# Autodesk Inventor assembly: tower1
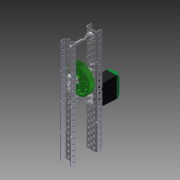
[picture p0: Inventor's stored thumbnail of the model, 180x180]
Saved by Autodesk Inventor 2014 SP1 (Build 180222100, 222)
## iProperties
Created: 2013-08-29
Part Number: tower1
Document SubType Name: Assembly
Designer: Ryan
Author: Ryan
## Documents named in this file (19)
- C:\Users\Ryan\Desktop\sw\toss up 1st A bot\toss up tower\tower1.iam
- C:\Users\Ryan\Desktop\sw\lib\Aperture VEX CAD Library\Metal\C Channel\2 x 20.ipt
- C:\Users\Ryan\Desktop\sw\lib\Aperture VEX CAD Library\Bearing Blocks\Bearing Block with screws.iam
- C:\Users\Ryan\Desktop\sw\lib\Aperture VEX CAD Library\Hardware\8-32\8-32_.375.ipt
- C:\Users\Ryan\Desktop\sw\lib\Aperture VEX CAD Library\Shaft\2 inch Shaft.ipt
- C:\Users\Ryan\Desktop\sw\lib\Aperture VEX CAD Library\Gears\High Strength Gears\60 Tooth Round Insert.iam
- C:\Users\Ryan\Desktop\sw\lib\Aperture VEX CAD Library\Gears\High Strength Gears\HS-GEAR-12TOOTH.ipt
- C:\Users\Ryan\Desktop\sw\lib\Super Sonic Sparks VEX CAD Library\Motors & Sensors\2-Wire Motor 393-Without Wire.iam
- C:\Users\Ryan\Desktop\sw\lib\Aperture VEX CAD Library\Bearing Blocks\Bearing Block.ipt
- C:\Users\Ryan\Desktop\sw\lib\Aperture VEX CAD Library\Hardware\6-32\6-32_.500.ipt
- C:\Users\Ryan\Desktop\sw\lib\Aperture VEX CAD Library\Shaft\3 inch Shaft.ipt
- C:\Users\Ryan\Desktop\sw\lib\Aperture VEX CAD Library\Spacers\SPACER-0500-0125.ipt
- C:\Users\Ryan\Desktop\sw\lib\Aperture VEX CAD Library\Spacers\SPACER-0500-0500.ipt
- C:\Users\Ryan\Desktop\sw\lib\Aperture VEX CAD Library\Spacers\SPACER-0500-0250.ipt
- C:\Users\Ryan\Desktop\sw\lib\Aperture VEX CAD Library\Hardware\Shaft Collar.ipt
- C:\Users\Ryan\Desktop\sw\lib\Aperture VEX CAD Library\Metal\0.5x12.5 inch Beam.ipt
- C:\Users\Ryan\Desktop\sw\lib\Imported Components\8-32 nylock\8-32 nylock.ipt
- C:\Users\Ryan\Desktop\sw\lib\Aperture VEX CAD Library\Hardware\8-32\8-32_1.500.ipt
- C:\Users\Ryan\Desktop\sw\lib\Aperture VEX CAD Library\Standoffs\BEAM-1000.ipt
## Components (31 placed, 18 different names)
1. 2 x 20:1 — Flush:1, Flush:3, Mate:33, Flush:4, Mate:87, Mate:88, Mate:89, Mate:90, Mate:91, Mate:98, Mate:101, Mate:102, Mate:103, Mate:104, Mate:117, Flush:7, Flush:8, Flush:10, Mate:131, Mate:134
2. 2 x 20:2 — Flush:4, Mate:34, Mate:35, Mate:40, Mate:41, Mate:44, Flush:9, Flush:10, Mate:120, Mate:127, Mate:128, Mate:129, Mate:141
3. 2-Wire Motor 393-Without Wire:1 [sub-assembly] — Mate:34, Mate:45, Mate:46, Mate:50
4. 0.5x12.5 inch Beam:1 — Mate:117, Flush:7, Flush:8, Flush:9
5. Bearing Block with screws:2 [sub-assembly] — Mate:100, Mate:101, Mate:102, Mate:103, Mate:104, Mate:105
6. 3 inch Shaft:1 — Mate:50, Mate:51, Mate:52, Mate:53, Mate:54
7. HS-GEAR-12TOOTH:1 — Rotation:1, Mate:53, Mate:54, Mate:106, Mate:118
8. Bearing Block:1 — Mate:35, Mate:36, Mate:37, Mate:42, Mate:43, Mate:51, Mate:52, Mate:107, Mate:108
9. 6-32_.500:1 — Mate:36, Mate:37, Mate:40, Mate:41, Mate:46
10. 6-32_.500:2 — Mate:42, Mate:43, Mate:44, Mate:45
11. SPACER-0500-0250:1 — Mate:100, Mate:105, Mate:106
12. SPACER-0500-0250:2 — Mate:107, Mate:108, Mate:114, Mate:115
13. SPACER-0500-0125:3 — Mate:114, Mate:115, Mate:116
14. Shaft Collar:1 — Mate:116, Mate:118
15. 8-32 nylock:1 — Mate:126, Mate:127, Mate:128, Mate:130
16. 8-32_1.500:1 — Mate:129, Mate:130, Mate:132, Mate:137, Mate:140
17. 8-32_.375:19 — Mate:131, Mate:132, Mate:133
18. BEAM-1000:1 — Mate:133, Mate:134
19. SPACER-0500-0250:4 — Mate:137, Mate:139, Mate:126
20. SPACER-0500-0125:4 — Mate:139, Mate:140, Mate:141
21. 2 inch Shaft:1 — Flush:1, Mate:94, Mate:95
22. 60 Tooth Round Insert:1 [sub-assembly] — Rotation:1, Mate:96, Mate:99
23. Bearing Block:2 — Mate:87, Mate:88, Mate:89, Mate:90, Mate:92, Mate:94, Mate:95, Mate:96, Mate:97
24. SPACER-0500-0500:1 — Mate:97, Mate:98, Mate:99, Mate:119
25. SPACER-0500-0250:3 — Mate:119, Mate:120, Mate:122, Mate:123
26. Shaft Collar:2 — Mate:122, Mate:123
27. Bearing Block:3 — Mate:143
28. 8-32_.375:20 — Mate:143
29. 8-32_.375:21
30. 8-32_.375:13 — Mate:91, Mate:92
31. 8-32_.375:14
## Component patterns: (2 elements, first: 8-32_.375:13)
## Relationships (70: Mate 62, Flush 7, RelateRotation 1)
- Flush:1: 2 x 20:1 ↔ 2 inch Shaft:1
- Flush:3 (24.2316 mm): 2 x 20:1
- Rotation:1 [RelateRotation] (0.2 ul): HS-GEAR-12TOOTH:1 ↔ 60 Tooth Round Insert:1
- Mate:33: 2 x 20:1
- Flush:4: 2 x 20:1 ↔ 2 x 20:2
- Mate:34: 2 x 20:2 ↔ 2-Wire Motor 393-Without Wire:1
- Mate:35: 2 x 20:2 ↔ Bearing Block:1
- Mate:36: Bearing Block:1 ↔ 6-32_.500:1
- Mate:37: Bearing Block:1 ↔ 6-32_.500:1
- Mate:40 (2.3114 mm): 2 x 20:2 ↔ 6-32_.500:1
- Mate:41 (2.3114 mm): 2 x 20:2 ↔ 6-32_.500:1
- Mate:42: Bearing Block:1 ↔ 6-32_.500:2
- Mate:43: Bearing Block:1 ↔ 6-32_.500:2
- Mate:44 (2.3114 mm): 2 x 20:2 ↔ 6-32_.500:2
- Mate:45: 2-Wire Motor 393-Without Wire:1 ↔ 6-32_.500:2
- Mate:46: 2-Wire Motor 393-Without Wire:1 ↔ 6-32_.500:1
- Mate:50: 2-Wire Motor 393-Without Wire:1 ↔ 3 inch Shaft:1
- Mate:51 (-1.5875 mm): 3 inch Shaft:1 ↔ Bearing Block:1
- Mate:52 (-1.5875 mm): 3 inch Shaft:1 ↔ Bearing Block:1
- Mate:53: 3 inch Shaft:1 ↔ HS-GEAR-12TOOTH:1
- Mate:54: 3 inch Shaft:1 ↔ HS-GEAR-12TOOTH:1
- Mate:87: 2 x 20:1 ↔ Bearing Block:2
- Mate:88 (2.3114 mm): 2 x 20:1 ↔ Bearing Block:2
- Mate:89 (2.3114 mm): 2 x 20:1 ↔ Bearing Block:2
- Mate:90 (2.3114 mm): 2 x 20:1 ↔ Bearing Block:2
- Mate:91: 2 x 20:1 ↔ 8-32_.375:13
- Mate:92: Bearing Block:2 ↔ 8-32_.375:13
- Mate:94 (-1.5875 mm): 2 inch Shaft:1 ↔ Bearing Block:2
- Mate:95 (-1.5875 mm): 2 inch Shaft:1 ↔ Bearing Block:2
- Mate:96: 60 Tooth Round Insert:1 ↔ Bearing Block:2
- Mate:97: Bearing Block:2 ↔ SPACER-0500-0500:1
- Mate:98: 2 x 20:1 ↔ SPACER-0500-0500:1
- Mate:99: 60 Tooth Round Insert:1 ↔ SPACER-0500-0500:1
- Mate:100: Bearing Block with screws:2 ↔ SPACER-0500-0250:1
- Mate:101: 2 x 20:1 ↔ Bearing Block with screws:2
- Mate:102 (2.3114 mm): 2 x 20:1 ↔ Bearing Block with screws:2
- Mate:103 (2.3114 mm): 2 x 20:1 ↔ Bearing Block with screws:2
- Mate:104 (2.3114 mm): 2 x 20:1 ↔ Bearing Block with screws:2
- Mate:105: Bearing Block with screws:2 ↔ SPACER-0500-0250:1
- Mate:106: HS-GEAR-12TOOTH:1 ↔ SPACER-0500-0250:1
- Mate:107: Bearing Block:1 ↔ SPACER-0500-0250:2
- Mate:108: Bearing Block:1 ↔ SPACER-0500-0250:2
- Mate:114: SPACER-0500-0250:2 ↔ SPACER-0500-0125:3
- Mate:115: SPACER-0500-0250:2 ↔ SPACER-0500-0125:3
- Mate:116: SPACER-0500-0125:3 ↔ Shaft Collar:1
- Mate:117: 2 x 20:1 ↔ 0.5x12.5 inch Beam:1
- Flush:7: 2 x 20:1 ↔ 0.5x12.5 inch Beam:1
- Flush:8: 2 x 20:1 ↔ 0.5x12.5 inch Beam:1
- Flush:9: 2 x 20:2 ↔ 0.5x12.5 inch Beam:1
- Mate:118: HS-GEAR-12TOOTH:1 ↔ Shaft Collar:1
- Flush:10: 2 x 20:1 ↔ 2 x 20:2
- Mate:119: SPACER-0500-0500:1 ↔ SPACER-0500-0250:3
- Mate:120: 2 x 20:2 ↔ SPACER-0500-0250:3
- Mate:122: SPACER-0500-0250:3 ↔ Shaft Collar:2
- Mate:123: SPACER-0500-0250:3 ↔ Shaft Collar:2
- Mate:126: 8-32 nylock:1 ↔ SPACER-0500-0250:4
- Mate:127 (2.3114 mm): 2 x 20:2 ↔ 8-32 nylock:1
- Mate:128 (2.3114 mm): 2 x 20:2 ↔ 8-32 nylock:1
- Mate:129: 2 x 20:2 ↔ 8-32_1.500:1
- Mate:130: 8-32 nylock:1 ↔ 8-32_1.500:1
- Mate:131: 2 x 20:1 ↔ 8-32_.375:19
- Mate:132: 8-32_1.500:1 ↔ 8-32_.375:19
- Mate:133: 8-32_.375:19 ↔ BEAM-1000:1
- Mate:134: 2 x 20:1 ↔ BEAM-1000:1
- Mate:137: 8-32_1.500:1 ↔ SPACER-0500-0250:4
- Mate:139: SPACER-0500-0250:4 ↔ SPACER-0500-0125:4
- Mate:140: 8-32_1.500:1 ↔ SPACER-0500-0125:4
- Mate:141: 2 x 20:2 ↔ SPACER-0500-0125:4
- Mate:142
- Mate:143: Bearing Block:3 ↔ 8-32_.375:20
## Named parameters: q = 2.3114 mm, sh = -1.5875 mm
